# Autodesk Inventor assembly: Assembly1
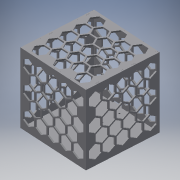
[picture p0: Inventor's stored thumbnail of the model, 180x180]
Saved by Autodesk Inventor 2019 (Build 230136000, 136)
## iProperties
Created: 2019-04-06
Part Number: Assembly1
Document SubType Name: Assembly
Designer: Daniel
Author: Daniel
## Documents named in this file (5)
- E:\Projekte\LichtWuefel\Assembly1.iam
- E:\Projekte\LichtWuefel\Part1.ipt
- E:\Projekte\LichtWuefel\TOP.ipt
- E:\Projekte\LichtWuefel\bot.ipt
- E:\Projekte\LichtWuefel\back2.ipt
## Components (6 placed, 4 different names)
1. Part1:1 — Rigid:2
2. Part1:2 — Rigid:3
3. Part1:3 — Rigid:1, Rigid:5
4. TOP:1 — Rigid:5
5. bot:1 — Rigid:1, Rigid:2, Rigid:3, Rigid:4
6. back2:1 — Rigid:4
## Relationships (5: WeldJoint 5)
- Rigid:1 [WeldJoint]: Part1:3 ↔ bot:1
- Rigid:2 [WeldJoint]: Part1:1 ↔ bot:1
- Rigid:3 [WeldJoint]: Part1:2 ↔ bot:1
- Rigid:4 [WeldJoint]: bot:1 ↔ back2:1
- Rigid:5 [WeldJoint]: Part1:3 ↔ TOP:1
